# Autodesk Inventor assembly: ForearmActuatorShaft
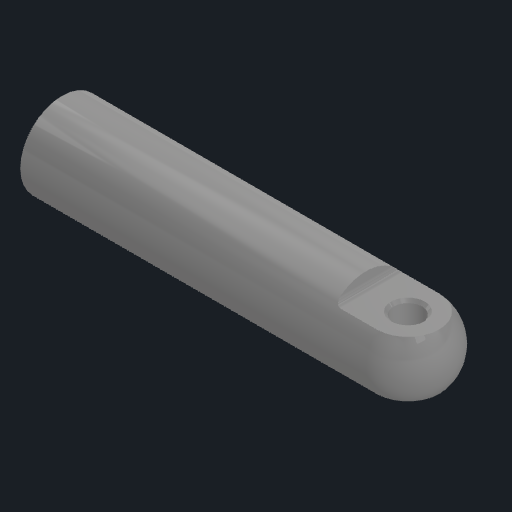
[picture p0: Inventor's stored thumbnail of the model, 512x512]
Saved by Autodesk Inventor 2023 (Build 270158000, 158)
## iProperties
Created: 2023-03-25
Part Number: ForearmActuatorShaft
Document SubType Name: Assembly
Designer: Val
Author: Val
## Documents named in this file (3)
- C:\Users\valer\Desktop\str1ker\cad\external\ForearmActuator\ForearmActuatorShaft.iam
- C:\Users\valer\Desktop\str1ker\cad\external\ForearmActuator\ForearmActuatorShaft.ipt
- C:\Users\valer\Desktop\str1ker\cad\external\ForearmActuator\ForearmActuatorBodyBoundingBox.ipt
## Components (2 placed, 2 different names)
1. ForearmActuatorShaft:1 — Mate:1, Angle:1, Angle:2, Flush:2
2. ForearmActuatorBodyBoundingBox:1 — Flush:1, Mate:2, Flush:2
## Relationships (6: Mate 2, Flush 2, Angle 2)
- Mate:1: ForearmActuatorShaft:1
- Flush:1: ForearmActuatorBodyBoundingBox:1
- Angle:1 (180 deg): ForearmActuatorShaft:1
- Angle:2 (0 deg): ForearmActuatorShaft:1
- Mate:2: ForearmActuatorBodyBoundingBox:1
- Flush:2: ForearmActuatorShaft:1 ↔ ForearmActuatorBodyBoundingBox:1
